# Autodesk Inventor assembly: FirstIntakes
(part 3 of 3)
- Angle:302 (0 deg): 1 x 1 x 0.040 x 14 Intake Pre-Drilled VersaFrame Aluminum Tube Stock Cut Modified (217-3426):1 ↔ #8-32 x 2.000 Star Drive Screw (276-8015):43
- Angle:303 (0 deg): 1 x 1 x 0.040 x 14 Intake Pre-Drilled VersaFrame Aluminum Tube Stock Cut Modified (217-3426):1 ↔ #8-32 x 2.000 Star Drive Screw (276-8015):60
- Angle:304 (0 deg): 1 x 1 x 0.040 x 14 Intake Pre-Drilled VersaFrame Aluminum Tube Stock Cut Modified (217-3426):1 ↔ #8-32 x 2.000 Star Drive Screw (276-8015):59
- Angle:305 (0 deg): 1 x 1 x 0.040 x 14 Intake Pre-Drilled VersaFrame Aluminum Tube Stock Cut Modified (217-3426):1 ↔ #8-32 x 2.000 Star Drive Screw (276-8015):58
- Angle:306 (0 deg): 1 x 1 x 0.040 x 14 Intake Pre-Drilled VersaFrame Aluminum Tube Stock Cut Modified (217-3426):1 ↔ #8-32 x 2.000 Star Drive Screw (276-8015):57
- Angle:307 (0 deg): 1 x 1 x 0.040 x 14 Intake Pre-Drilled VersaFrame Aluminum Tube Stock Cut Modified (217-3426):1 ↔ #8-32 x 2.000 Star Drive Screw (276-8015):56
- Angle:308 (0 deg): 1 x 1 x 0.040 x 14 Intake Pre-Drilled VersaFrame Aluminum Tube Stock Cut Modified (217-3426):1 ↔ #8-32 x 2.000 Star Drive Screw (276-8015):55
- Angle:309 (0 deg): 1 x 1 x 0.040 x 14 Intake Pre-Drilled VersaFrame Aluminum Tube Stock Cut Modified (217-3426):1 ↔ #8-32 x 2.000 Star Drive Screw (276-8015):54
- Angle:310 (0 deg): 1 x 1 x 0.040 x 14 Intake Pre-Drilled VersaFrame Aluminum Tube Stock Cut Modified (217-3426):1 ↔ #8-32 x 2.000 Star Drive Screw (276-8015):53
- Angle:311 (0 deg): 1 x 1 x 0.040 x 14 Intake Pre-Drilled VersaFrame Aluminum Tube Stock Cut Modified (217-3426):1 ↔ #8-32 x 2.000 Star Drive Screw (276-8015):52
- Angle:312 (0 deg): 1 x 1 x 0.040 x 14 Intake Pre-Drilled VersaFrame Aluminum Tube Stock Cut Modified (217-3426):1 ↔ #8-32 x 2.000 Star Drive Screw (276-8015):51
- Angle:313 (0 deg): 1 x 1 x 0.040 x 14 Intake Pre-Drilled VersaFrame Aluminum Tube Stock Cut Modified (217-3426):1 ↔ #8-32 x 2.000 Star Drive Screw (276-8015):50
- Angle:314 (0 deg): 1 x 1 x 0.040 x 14 Intake Pre-Drilled VersaFrame Aluminum Tube Stock Cut Modified (217-3426):1 ↔ #8-32 x 2.000 Star Drive Screw (276-8015):49
- Mate:712: 13.75mm (1_2 ThunderHex ID) x 1.125 OD x 0.313 WD (Flanged Bearing) (217-4006):1 ↔ 1_2 Hex x 0.201 x 10.5 ID ThunderHex Stock Cut (217-4017):1
- Mate:713: 13.75mm (1_2 ThunderHex ID) x 1.125 OD x 0.313 WD (Flanged Bearing) (217-4006):2 ↔ 1_2 Hex x 0.201 x 10.5 ID ThunderHex Stock Cut (217-4017):2
- Angle:315 (0 deg): Clamping Shaft Collar - 1_2 Hex ID (217-2737):6 ↔ 1_2 Hex x 0.201 x 10.5 ID ThunderHex Stock Cut (217-4017):2
- Angle:316 (0 deg): Clamping Shaft Collar - 1_2 Hex ID (217-2737):7 ↔ 1_2 Hex x 0.201 x 10.5 ID ThunderHex Stock Cut (217-4017):1
- Flush:561 (-2.54 mm): 13.75mm (1_2 ThunderHex ID) x 1.125 OD x 0.313 WD (Flanged Bearing) (217-4006):2 ↔ 1_2 Hex x 0.201 x 10.5 ID ThunderHex Stock Cut (217-4017):2
- Flush:562 (-3.81 mm): 13.75mm (1_2 ThunderHex ID) x 1.125 OD x 0.313 WD (Flanged Bearing) (217-4006):1 ↔ 1_2 Hex x 0.201 x 10.5 ID ThunderHex Stock Cut (217-4017):1
- Mate:714: VersaPlanetary v2 One Stage Universal Output:1 ↔ Falcon 500, Powered by Talon FX (217-6515):1
- Mate:715: VersaPlanetary v2 One Stage Universal Output:1 ↔ Falcon 500, Powered by Talon FX (217-6515):1
- Mate:716: VersaPlanetary v2 One Stage Universal Output:1 ↔ Falcon 500, Powered by Talon FX (217-6515):1
- Mate:717: 13.75mm (1_2 ThunderHex ID) x 1.125 OD x 0.313 WD (Flanged Bearing) (217-4006):11 ↔ 1_2 Hex x 0.201 x 11 ID ThunderHex Stock Cut (217-4017):1
- Angle:317 (0 deg): 1 x 1 x 0.040 x 14 Intake Pre-Drilled VersaFrame Aluminum Tube Stock Cut Modified (217-3426):1 ↔ 1_2 Hex x 0.201 x 11 ID ThunderHex Stock Cut (217-4017):1
- Mate:718: VersaPlanetary v2 One Stage Universal Output:1 ↔ 1_2 Hex x 0.201 x 11 ID ThunderHex Stock Cut (217-4017):1
- Flush:563 (-127 mm): 1 x 1 x 0.040 x 14 Intake Pre-Drilled VersaFrame Aluminum Tube Stock Cut Modified (217-3426):1
- Mate:719 (127 mm): 1 x 1 x 0.040 x 14 Intake Pre-Drilled VersaFrame Aluminum Tube Stock Cut Modified (217-3426):2
- Mate:720: 13.75mm (1_2 ThunderHex ID) x 1.125 OD x 0.313 WD (Flanged Bearing) (217-4006):9 ↔ 1_2 Acetal Spacer - 1_2 Hex (217-2758):8
- Mate:721: 13.75mm (1_2 ThunderHex ID) x 1.125 OD x 0.313 WD (Flanged Bearing) (217-4006):9 ↔ 1_2 Acetal Spacer - 1_2 Hex (217-2758):8
- Angle:318 (0 deg): 1_2 Acetal Spacer - 1_2 Hex (217-2758):5 ↔ 1_2 Acetal Spacer - 1_2 Hex (217-2758):8
- Angle:319 (0 deg): 1_2 Acetal Spacer - 1_2 Hex (217-2758):6 ↔ 1_2 Acetal Spacer - 1_2 Hex (217-2758):9
- Mate:722: 13.75mm (1_2 ThunderHex ID) x 1.125 OD x 0.313 WD (Flanged Bearing) (217-4006):7 ↔ 1_2 Acetal Spacer - 1_2 Hex (217-2758):9
- Mate:723: 13.75mm (1_2 ThunderHex ID) x 1.125 OD x 0.313 WD (Flanged Bearing) (217-4006):7 ↔ 1_2 Acetal Spacer - 1_2 Hex (217-2758):9
- Mate:724: 13.75mm (1_2 ThunderHex ID) x 1.125 OD x 0.313 WD (Flanged Bearing) (217-4006):8 ↔ Clamping Shaft Collar - 1_2 Hex ID (217-2737):16
- Angle:320 (0 deg): 1_8 Acetal Spacer - 1_2 Hex (217-2758):1 ↔ Clamping Shaft Collar - 1_2 Hex ID (217-2737):16
- Mate:725: 13.75mm (1_2 ThunderHex ID) x 1.125 OD x 0.313 WD (Flanged Bearing) (217-4006):8 ↔ Clamping Shaft Collar - 1_2 Hex ID (217-2737):16
- Angle:321 (0 deg): 1_2 Acetal Spacer - 1_2 Hex (217-2758):6 ↔ Clamping Shaft Collar - 1_2 Hex ID (217-2737):17
- Mate:726: 13.75mm (1_2 ThunderHex ID) x 1.125 OD x 0.313 WD (Flanged Bearing) (217-4006):10 ↔ Clamping Shaft Collar - 1_2 Hex ID (217-2737):17
- Mate:727: 13.75mm (1_2 ThunderHex ID) x 1.125 OD x 0.313 WD (Flanged Bearing) (217-4006):10 ↔ Clamping Shaft Collar - 1_2 Hex ID (217-2737):17
- Angle:322 (0 deg): 1_2 Acetal Spacer - 1_2 Hex (217-2758):8 ↔ 1_2 Hex x 0.201 x 4 ID ThunderHex Stock Cut (217-4017):1
- Angle:323 (0 deg): Clamping Shaft Collar - 1_2 Hex ID (217-2737):17 ↔ 1_2 Hex x 0.201 x 4 ID ThunderHex Stock Cut (217-4017):2
- Flush:564: Clamping Shaft Collar - 1_2 Hex ID (217-2737):17 ↔ 1_2 Hex x 0.201 x 4 ID ThunderHex Stock Cut (217-4017):2
- Flush:565: Clamping Shaft Collar - 1_2 Hex ID (217-2737):16 ↔ 1_2 Hex x 0.201 x 4 ID ThunderHex Stock Cut (217-4017):1
- Mate:728: Clamping Shaft Collar - 1_2 Hex ID (217-2737):16 ↔ 1_2 Hex x 0.201 x 4 ID ThunderHex Stock Cut (217-4017):1
- Mate:729: Clamping Shaft Collar - 1_2 Hex ID (217-2737):17 ↔ 1_2 Hex x 0.201 x 4 ID ThunderHex Stock Cut (217-4017):2
- Mate:730: 5.00 Standoff  (275-1022):1 ↔ #8-32 x 1.000 Star Drive Coupler (276-4988):1
- Mate:731: 5.00 Standoff  (275-1022):2 ↔ #8-32 x 1.000 Star Drive Coupler (276-4988):1
- Angle:324 (0 deg): 5.00 Standoff  (275-1022):1 ↔ 5.00 Standoff  (275-1022):2
- Mate:732: 5.00 Standoff  (275-1022):1 ↔ #8-32 x 1.000 Star Drive Coupler (276-4988):1
- Mate:733: 5.00 Standoff  (275-1022):1 ↔ 5.00 Standoff  (275-1022):2
- Angle:325 (0 deg): 5.00 Standoff  (275-1022):2 ↔ #8-32 x 1.000 Star Drive Coupler (276-4988):1
- [Mate]: 5.00 Standoff  (275-1022):3 ↔ #8-32 x 1.000 Star Drive Coupler (276-4988):2
- [Mate]: 5.00 Standoff  (275-1022):4 ↔ #8-32 x 1.000 Star Drive Coupler (276-4988):2
- [Angle] (0 deg): 5.00 Standoff  (275-1022):3 ↔ 5.00 Standoff  (275-1022):4
- [Mate]: 5.00 Standoff  (275-1022):3 ↔ #8-32 x 1.000 Star Drive Coupler (276-4988):2
- [Mate]: 5.00 Standoff  (275-1022):3 ↔ 5.00 Standoff  (275-1022):4
- Angle:327 (0 deg): 5.00 Standoff  (275-1022):4 ↔ #8-32 x 1.000 Star Drive Coupler (276-4988):2
- Angle:328 (0 deg): 1 x 1 x 0.040 x 14 Intake Pre-Drilled VersaFrame Aluminum Tube Stock Cut Modified (217-3426):2 ↔ 5.00 Standoff  (275-1022):3
- Angle:329 (0 deg): 1 x 1 x 0.040 x 14 Intake Pre-Drilled VersaFrame Aluminum Tube Stock Cut Modified (217-3426):2 ↔ 5.00 Standoff  (275-1022):1
- Mate:738: 1 x 1 x 0.040 x 14 Intake Pre-Drilled VersaFrame Aluminum Tube Stock Cut Modified (217-3426):2 ↔ 5.00 Standoff  (275-1022):1
- Mate:739: 1 x 1 x 0.040 x 14 Intake Pre-Drilled VersaFrame Aluminum Tube Stock Cut Modified (217-3426):2 ↔ 5.00 Standoff  (275-1022):3
- Mate:740: 1 x 1 x 0.040 x 14 Intake Pre-Drilled VersaFrame Aluminum Tube Stock Cut Modified (217-3426):2 ↔ 5.00 Standoff  (275-1022):1
- Mate:741: 1 x 1 x 0.040 x 14 Intake Pre-Drilled VersaFrame Aluminum Tube Stock Cut Modified (217-3426):2 ↔ 5.00 Standoff  (275-1022):3
- Mate:742: 1 x 1 x 0.040 x 14 Intake Pre-Drilled VersaFrame Aluminum Tube Stock Cut Modified (217-3426):1 ↔ #8-32 x 1.500 Star Drive Screw (276-4998):19
- Mate:743: 1 x 1 x 0.040 x 14 Intake Pre-Drilled VersaFrame Aluminum Tube Stock Cut Modified (217-3426):1 ↔ #8-32 x 1.500 Star Drive Screw (276-4998):20
- Mate:744: 1 x 1 x 0.040 x 14 Intake Pre-Drilled VersaFrame Aluminum Tube Stock Cut Modified (217-3426):1 ↔ #8-32 x 1.500 Star Drive Screw (276-4998):19
- Mate:745: 1 x 1 x 0.040 x 14 Intake Pre-Drilled VersaFrame Aluminum Tube Stock Cut Modified (217-3426):1 ↔ #8-32 x 1.500 Star Drive Screw (276-4998):20
- Mate:746: 1 x 1 x 0.040 x 14 Intake Pre-Drilled VersaFrame Aluminum Tube Stock Cut Modified (217-3426):2 ↔ #8-32 x 1.500 Star Drive Screw (276-4998):18
- Mate:747: 1 x 1 x 0.040 x 14 Intake Pre-Drilled VersaFrame Aluminum Tube Stock Cut Modified (217-3426):2 ↔ #8-32 x 1.500 Star Drive Screw (276-4998):17
- Mate:748: 1 x 1 x 0.040 x 14 Intake Pre-Drilled VersaFrame Aluminum Tube Stock Cut Modified (217-3426):2 ↔ #8-32 x 1.500 Star Drive Screw (276-4998):17
- Mate:749: 1 x 1 x 0.040 x 14 Intake Pre-Drilled VersaFrame Aluminum Tube Stock Cut Modified (217-3426):2 ↔ #8-32 x 1.500 Star Drive Screw (276-4998):18
- Angle:330 (0 deg): 1 x 1 x 0.040 x 14 Intake Pre-Drilled VersaFrame Aluminum Tube Stock Cut Modified (217-3426):1 ↔ #8-32 x 1.500 Star Drive Screw (276-4998):20
- Angle:331 (0 deg): 1 x 1 x 0.040 x 14 Intake Pre-Drilled VersaFrame Aluminum Tube Stock Cut Modified (217-3426):1 ↔ #8-32 x 1.500 Star Drive Screw (276-4998):19
- Angle:332 (0 deg): 1 x 1 x 0.040 x 14 Intake Pre-Drilled VersaFrame Aluminum Tube Stock Cut Modified (217-3426):2 ↔ #8-32 x 1.500 Star Drive Screw (276-4998):18
- Angle:333 (0 deg): 1 x 1 x 0.040 x 14 Intake Pre-Drilled VersaFrame Aluminum Tube Stock Cut Modified (217-3426):2 ↔ #8-32 x 1.500 Star Drive Screw (276-4998):17
- Mate:750: 1 x 1 x 0.040 x 14 Intake Pre-Drilled VersaFrame Aluminum Tube Stock Cut Modified (217-3426):2 ↔ 2.00 Standoff  (275-1018):1
- Mate:751: 1 x 1 x 0.040 x 14 Intake Pre-Drilled VersaFrame Aluminum Tube Stock Cut Modified (217-3426):2 ↔ 2.00 Standoff  (275-1018):1
- Angle:334 (0 deg): 1 x 1 x 0.040 x 14 Intake Pre-Drilled VersaFrame Aluminum Tube Stock Cut Modified (217-3426):2 ↔ 2.00 Standoff  (275-1018):1
- Angle:335 (0 deg): 1 x 1 x 0.040 x 14 Intake Pre-Drilled VersaFrame Aluminum Tube Stock Cut Modified (217-3426):1 ↔ 2.00 Standoff  (275-1018):2
- Mate:752: 1 x 1 x 0.040 x 14 Intake Pre-Drilled VersaFrame Aluminum Tube Stock Cut Modified (217-3426):1 ↔ 2.00 Standoff  (275-1018):2
- Mate:753: 1 x 1 x 0.040 x 14 Intake Pre-Drilled VersaFrame Aluminum Tube Stock Cut Modified (217-3426):1 ↔ 2.00 Standoff  (275-1018):2
- Mate:754: 1 x 1 x 0.040 x 14 Intake Pre-Drilled VersaFrame Aluminum Tube Stock Cut Modified (217-3426):1 ↔ #8-32 x 1.500 Star Drive Screw (276-4998):22
- Mate:755: 1 x 1 x 0.040 x 14 Intake Pre-Drilled VersaFrame Aluminum Tube Stock Cut Modified (217-3426):2 ↔ #8-32 x 1.500 Star Drive Screw (276-4998):21
- Mate:756: 1 x 1 x 0.040 x 14 Intake Pre-Drilled VersaFrame Aluminum Tube Stock Cut Modified (217-3426):2 ↔ #8-32 x 1.500 Star Drive Screw (276-4998):21
- Mate:757: 1 x 1 x 0.040 x 14 Intake Pre-Drilled VersaFrame Aluminum Tube Stock Cut Modified (217-3426):1 ↔ #8-32 x 1.500 Star Drive Screw (276-4998):22
- Angle:336 (0 deg): 1 x 1 x 0.040 x 14 Intake Pre-Drilled VersaFrame Aluminum Tube Stock Cut Modified (217-3426):2 ↔ #8-32 x 1.500 Star Drive Screw (276-4998):21
- Angle:337 (0 deg): 1 x 1 x 0.040 x 14 Intake Pre-Drilled VersaFrame Aluminum Tube Stock Cut Modified (217-3426):1 ↔ #8-32 x 1.500 Star Drive Screw (276-4998):22
- Mate:758: VersaPlanetary v2 One Stage Universal Output:1 ↔ CIM Motor (217-2000):1
- Mate:759: VersaPlanetary v2 One Stage Universal Output:1 ↔ CIM Motor (217-2000):1
- Mate:760: VersaPlanetary v2 One Stage Universal Output:1 ↔ CIM Motor (217-2000):1
## Named parameters: d165_d38 = 0 mm, d166_d41 = 0 mm, d167_d44 = 0 mm, d168_d27 = 0 mm, d169_d28 = 0 mm, d170_d33 = 0 mm, d171_d106 = 0 mm, d178_d148 = 0 deg, d179_d149 = 0 deg, d180_d150 = 0 deg, d181_d151 = 0 deg, d182_d152 = 0 deg, d183_d153 = 0 deg, d184_d154 = 0 mm, d185_d118 = 0 mm, d186_d119 = 0 mm, d187_d120 = 0 mm, d188_d121 = 0 mm, d189_d122 = 0 mm, d190_d123 = 0 mm, d191_d124 = 0 mm, d192_d125 = 0 mm, d193_d126 = 0 mm, d194_d127 = 0 mm, d195_d128 = 0 mm, d196_d129 = 0 mm, d209_d155 = 0 deg, d210_d156 = 0 mm, d211_d157 = 0 deg, d212_d158 = 0 mm, d213_d159 = 0 deg, d214_d160 = 0 mm, d215_d161 = 0 mm, d216_d162 = 0 mm, d217_d163 = 0 deg, d218_d164 = 0 mm, d219_d38 = 0 mm, d220_d41 = 0 mm, d221_d44 = 0 mm, d222_d27 = 0 mm, d223_d28 = 0 mm, d224_d33 = 0 mm, d238_d154 = 0 mm, d239_d118 = 0 mm, d240_d119 = 0 mm, d241_d120 = 0 mm, d242_d121 = 0 mm, d243_d122 = 0 mm, d244_d123 = 0 mm, d245_d124 = 0 mm, d246_d125 = 0 mm, d247_d126 = 0 mm, d248_d127 = 0 mm, d249_d128 = 0 mm, d250_d129 = 0 mm, d263_d155 = 0 deg, d264_d156 = 0 mm, d267_d159 = 0 deg, d268_d160 = 0 mm, d269_d161 = 0 mm, d270_d162 = 0 mm, d271_d163 = 0 deg, d272_d164 = 0 mm, d273_d38 = 0 mm, d274_d41 = 0 mm, d275_d44 = 0 mm, d276_d27 = 0 mm, d277_d28 = 0 mm, d278_d33 = 0 mm, d280_d142 = 0 deg, d281_d143 = 0 deg, d282_d144 = 0 deg, d283_d145 = 0 deg, d284_d146 = 0 deg, d285_d147 = 0 deg, d292_d154 = 0 mm, d293_d118 = 0 mm, d294_d119 = 0 mm, d295_d120 = 0 mm, d296_d121 = 0 mm, d297_d122 = 0 mm, d298_d123 = 0 mm, d299_d124 = 0 mm, d300_d125 = 0 mm, d301_d126 = 0 mm, d302_d127 = 0 mm, d303_d128 = 0 mm, d304_d129 = 0 mm, d305_d130 = 0 mm, d306_d131 = 0 mm, d307_d132 = 0 mm, d308_d133 = 0 mm, d309_d134 = 0 mm, d310_d135 = 0 mm, d311_d136 = 0 mm, d312_d137 = 0 mm, d313_d138 = 0 mm, d314_d139 = 0 mm, d315_d140 = 0 mm, d316_d141 = 0 mm, d317_d155 = 0 deg, d318_d156 = 0 mm, d453_d278_d33 = 0 mm, d454_d280_d142 = 0 deg, d455_d281_d143 = 0 deg, d456_d282_d144 = 0 deg, d457_d283_d145 = 0 deg, d458_d284_d146 = 0 deg, d459_d285_d147 = 0 deg, d461_d293_d118 = 0 mm, d462_d294_d119 = 0 mm, d463_d295_d120 = 0 mm, d464_d296_d121 = 0 mm, d465_d297_d122 = 0 mm, d466_d298_d123 = 0 mm, d467_d299_d124 = 0 mm, d468_d300_d125 = 0 mm, d469_d301_d126 = 0 mm, d470_d302_d127 = 0 mm, d471_d303_d128 = 0 mm, d472_d304_d129 = 0 mm, d473_d305_d130 = 0 mm, d474_d306_d131 = 0 mm, d475_d307_d132 = 0 mm, d476_d308_d133 = 0 mm, d477_d309_d134 = 0 mm, d478_d310_d135 = 0 mm, d479_d311_d136 = 0 mm, d480_d312_d137 = 0 mm, d481_d313_d138 = 0 mm, d482_d314_d139 = 0 mm, d483_d315_d140 = 0 mm, d484_d316_d141 = 0 mm, d487_d321_d159 = 0 deg, d489_d323_d161 = 0 mm, d490_d273_d38 = 0 mm, d491_d274_d41 = 0 mm, d492_d275_d44 = 0 mm, d493_d276_d27 = 0 mm, d494_d277_d28 = 0 mm, d495_d278_d33 = 0 mm, d496_d280_d142 = 0 deg, d497_d281_d143 = 0 deg, d498_d282_d144 = 0 deg, d499_d283_d145 = 0 deg, d500_d284_d146 = 0 deg, d501_d285_d147 = 0 deg, d502_d292_d154 = 0 mm, d503_d293_d118 = 0 mm, d504_d294_d119 = 0 mm, d505_d295_d120 = 0 mm, d506_d296_d121 = 0 mm, d507_d297_d122 = 0 mm, d508_d298_d123 = 0 mm, d509_d299_d124 = 0 mm, d510_d300_d125 = 0 mm, d511_d301_d126 = 0 mm, d512_d302_d127 = 0 mm, d513_d303_d128 = 0 mm, d514_d304_d129 = 0 mm, d515_d305_d130 = 0 mm, d516_d306_d131 = 0 mm, d517_d307_d132 = 0 mm, d518_d308_d133 = 0 mm, d519_d309_d134 = 0 mm, d520_d310_d135 = 0 mm, d521_d311_d136 = 0 mm, d522_d312_d137 = 0 mm, d523_d313_d138 = 0 mm, d524_d314_d139 = 0 mm, d525_d315_d140 = 0 mm, d526_d316_d141 = 0 mm, d527_d317_d155 = 0 deg, d528_d318_d156 = 0 mm, d532_d273_d38 = 0 mm, d533_d274_d41 = 0 mm, d534_d275_d44 = 0 mm, d535_d276_d27 = 0 mm, d536_d277_d28 = 0 mm, d545_d278_d33 = 0 mm, d546_d280_d142 = 0 deg, d547_d281_d143 = 0 deg, d548_d282_d144 = 0 deg, d549_d283_d145 = 0 deg, d550_d284_d146 = 0 deg, d551_d285_d147 = 0 deg, d553_d293_d118 = 0 mm, d554_d294_d119 = 0 mm, d555_d295_d120 = 0 mm, d556_d296_d121 = 0 mm, d557_d297_d122 = 0 mm, d558_d298_d123 = 0 mm, d559_d299_d124 = 0 mm, d560_d300_d125 = 0 mm, d561_d301_d126 = 0 mm, d562_d302_d127 = 0 mm, d563_d303_d128 = 0 mm, d564_d304_d129 = 0 mm, d565_d305_d130 = 0 mm, d566_d306_d131 = 0 mm, d567_d307_d132 = 0 mm, d568_d308_d133 = 0 mm, d569_d309_d134 = 0 mm, d570_d310_d135 = 0 mm, d571_d311_d136 = 0 mm, d572_d312_d137 = 0 mm, d573_d313_d138 = 0 mm, d574_d314_d139 = 0 mm, d575_d315_d140 = 0 mm, d576_d316_d141 = 0 mm, d579_d273_d38 = 0 mm, d580_d274_d41 = 0 mm, d581_d275_d44 = 0 mm, d582_d276_d27 = 0 mm, d583_d277_d28 = 0 mm, d818_d765 = 0 mm, d821_d735 = 0 mm, d822_d736 = 0 mm, d823_d737 = 0 mm, d824_d738 = 0 mm, d825_d739 = 0 mm, d826_d740 = 0 mm, d827_d741 = 0 mm, d828_d743 = 0 mm, d829_d744 = 0 mm, d833_d748 = 0 deg, d834_d749 = 0 deg, d835_d750 = 0 deg, d836_d751 = 0 deg, d837_d752 = 0 deg, d838_d753 = 0 deg, d839_d754 = 0 deg, d840_d755 = 0 deg, d841_d756 = 0 deg, d842_d757 = 0 deg, d843_d758 = 0 deg, d844_d759 = 0 deg, d845_d760 = 0 deg, d846_d761 = 0 deg, d847_d762 = 0 deg, d848_d763 = 0 deg, d849_d764 = 0 mm, d850_d716 = 0 mm, d851_d717 = 0 mm, d852_d718 = 0 mm, d853_d719 = 0 mm, d854_d720 = 0 mm, d855_d721 = 0 mm, d856_d722 = 0 mm, d857_d723 = 0 mm, d858_d724 = 0 mm, d859_d725 = 0 mm, d860_d726 = 0 mm, d861_d727 = 0 mm, d862_d728 = 0 mm, d864_d730 = 0 mm, d865_d731 = 0 mm, d866_d732 = 0 mm, d867_d733 = 0 mm, d868_d734 = 0 mm, d871_d7 = 0 mm, d872_d8 = 0 mm, d873_d9 = 0 mm, d875_d11 = 0 mm, d876_d12 = 0 mm, d879_d15 = 0 mm, d880_d16 = 0 mm, d882_d21 = 0 deg, d883_d22 = 0 deg, d887_d3 = 0 mm, d888_d4 = 0 mm, d927_d908 = 0 mm, d990_d926 = 0 mm, d991_d927 = 0 mm, d992_d928 = 0 mm, d993_d929 = 0 mm, d994_d930 = 0 deg, d995_d931 = 0 deg, d954_d990_d926 = 0 mm, d955_d991_d927 = 0 mm, d956_d992_d928 = 0 mm, d957_d993_d929 = 0 mm, d958_d994_d930 = 0 deg, d959_d995_d931 = 0 deg, d987_d954_d990_d926 = 0 mm, d988_d955_d991_d927 = 0 mm, d989_d956_d992_d928 = 0 mm, d990_d957_d993_d929 = 0 mm, d991_d958_d994_d930 = 0 deg, d992_d959_d995_d931 = 0 deg, d993_d962 = 0 mm, d994_d963 = 0 mm, d995_d927_d908 = 0 mm, d996_d928 = 0 mm, d997_d929 = 0 mm, d998_d930 = 0 mm, d999_d931 = 0 mm, d1000_d932 = 0 mm, d1001_d936 = 0 mm, d1002_d937 = 0 mm, d1003_d938 = 0 mm, d1004_d939 = 0 mm, d1092_d1086 = 0 mm, d1093_d1087 = 0 mm, d1094_d1088 = 0 deg, d1095_d1089 = 0 mm, d1096_d1090 = 0 mm, d1097_d1091 = 0 deg
